# Autodesk Inventor assembly: drivetrain
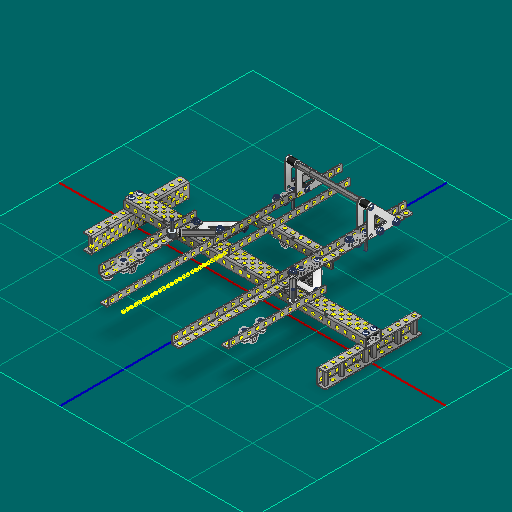
[picture p0: Inventor's stored thumbnail of the model, 512x512]
Saved by Autodesk Inventor 2025 (Build 290162000, 162)
## iProperties
Created: 2024-08-16
Part Number: drivetrain
Document SubType Name: Assembly
Designer: averey
Author: averey
## Documents named in this file (20)
- C:\Users\avere\vex_robotics_high_stakes\hardware\cad\ATLAS\chassis\structure\!structure.iam
- !structure.iam
- C:\Users\avere\vex_robotics_high_stakes\hardware\cad\ATLAS\chassis\structure\side_channel.iam
- C:\Users\avere\vex_robotics_high_stakes\hardware\cad\VEX-CAD-Inventor\Structure\Angle\Aluminum 1x1\Alu Angle 1x1x28.ipt
- C:\Users\avere\vex_robotics_high_stakes\hardware\cad\VEX-CAD-Inventor\Structure\C Channel\Aluminum 1x2x1\Alu C 1x2x1x30.ipt
- C:\Users\avere\vex_robotics_high_stakes\hardware\cad\ATLAS\chassis\structure\rail.iam
- C:\Users\avere\vex_robotics_high_stakes\hardware\cad\ATLAS\chassis\structure\rail_mirrored\rail_mirrored.iam
- C:\Users\avere\vex_robotics_high_stakes\hardware\cad\VEX-CAD-Inventor\Structure\Angle\Aluminum 1x1\Alu Angle 1x1x10.ipt
- C:\Users\avere\vex_robotics_high_stakes\hardware\cad\VEX-CAD-Inventor\Motion\Shaft LS\LS Pillow Bearing Block.ipt
- C:\Users\avere\vex_robotics_high_stakes\hardware\cad\VEX-CAD-Inventor\Motion\Spacers\Spacer Nylon .375 OD\NSpacer .375 OD x .375.ipt
- C:\Users\avere\vex_robotics_high_stakes\hardware\cad\VEX-CAD-Inventor\Motion\Spacers\Spacer Nylon .375 OD.ipt
- C:\Users\avere\vex_robotics_high_stakes\hardware\cad\VEX-CAD-Inventor\Motion\Spacers\Washer Teflon\TWasher .375 OD x .06250.ipt
- C:\Users\avere\vex_robotics_high_stakes\hardware\cad\VEX-CAD-Inventor\Motion\Spacers\Washer Teflon.ipt
- C:\Users\avere\vex_robotics_high_stakes\hardware\cad\VEX-CAD-Inventor\Structure\Hardware\Screw Steel - Star\SScrew Star Smooth .750.ipt
- C:\Users\avere\vex_robotics_high_stakes\hardware\cad\VEX-CAD-Inventor\Structure\Hardware\Screw Steel - Star.ipt
- C:\Users\avere\vex_robotics_high_stakes\hardware\cad\VEX-CAD-Inventor\Motion\Spacers\Spacer Nylon .500 OD\NSpacer White .500 OD x .125.ipt
- C:\Users\avere\vex_robotics_high_stakes\hardware\cad\VEX-CAD-Inventor\Motion\Spacers\Spacer Nylon .500 OD.ipt
- C:\Users\avere\vex_robotics_high_stakes\hardware\cad\VEX-CAD-Inventor\Structure\Standoff\Standoff .75.ipt
- C:\Users\avere\vex_robotics_high_stakes\hardware\cad\VEX-CAD-Inventor\Structure\Standoff.ipt
- C:\Users\avere\vex_robotics_high_stakes\hardware\cad\VEX-CAD-Inventor\Structure\Standoff\Standoff 3.00.ipt
## Components (19 placed, 13 different names)
1. side_channel:1 [sub-assembly] — Insert:83, Mate:44
2. side_channel:2 [sub-assembly] — Insert:82, Mate:43
3. Alu Angle 1x1x28:1
4. Alu C 1x2x1x30:1 — Insert:82, Mate:43, Insert:83, Mate:44, Insert:89, Mate:47, Insert:90, Mate:48, Mate:50, Insert:101, Insert:102, Insert:103, Insert:104
5. rail:1 [sub-assembly] — Insert:89, Mate:47, Mate:50, Mate:52, Insert:108
6. rail_mirrored:1 [sub-assembly] — Insert:90, Mate:48, Insert:92, Insert:105
7. Alu Angle 1x1x10:1 — Insert:92, Mate:52, Mate:53, Insert:100
8. LS Pillow Bearing Block:1 — Insert:98, Insert:99
9. NSpacer .375 OD x .375:1 — Insert:94, Insert:100
10. TWasher .375 OD x .06250:1 — Insert:94, Insert:99
11. TWasher .375 OD x .06250:2 — Insert:95, Insert:98
12. NSpacer .375 OD x .375:2 — Insert:95, Mate:53
13. SScrew Star Smooth .750:1 — Insert:101
14. SScrew Star Smooth .750:2 — Insert:102
15. SScrew Star Smooth .750:3 — Insert:103
16. SScrew Star Smooth .750:4 — Insert:104
17. NSpacer White .500 OD x .125:2 — Insert:105
18. Standoff .75:1 — Insert:107, Flush:1
19. Standoff 3.00:2 — Insert:107, Flush:1, Insert:108
## Relationships (25: Insert 17, Mate 7, Flush 1)
- Insert:82: side_channel:2 ↔ Alu C 1x2x1x30:1
- Mate:43: side_channel:2 ↔ Alu C 1x2x1x30:1
- Insert:83: side_channel:1 ↔ Alu C 1x2x1x30:1
- Mate:44: side_channel:1 ↔ Alu C 1x2x1x30:1
- Insert:89: Alu C 1x2x1x30:1 ↔ rail:1
- Mate:47: Alu C 1x2x1x30:1 ↔ rail:1
- Insert:90: Alu C 1x2x1x30:1 ↔ rail_mirrored:1
- Mate:48: Alu C 1x2x1x30:1 ↔ rail_mirrored:1
- Mate:50: Alu C 1x2x1x30:1 ↔ rail:1
- Insert:92: rail_mirrored:1 ↔ Alu Angle 1x1x10:1
- Mate:52: rail:1 ↔ Alu Angle 1x1x10:1
- Insert:94: NSpacer .375 OD x .375:1 ↔ TWasher .375 OD x .06250:1
- Insert:95: TWasher .375 OD x .06250:2 ↔ NSpacer .375 OD x .375:2
- Insert:98: LS Pillow Bearing Block:1 ↔ TWasher .375 OD x .06250:2
- Insert:99: LS Pillow Bearing Block:1 ↔ TWasher .375 OD x .06250:1
- Mate:53: Alu Angle 1x1x10:1 ↔ NSpacer .375 OD x .375:2
- Insert:100: Alu Angle 1x1x10:1 ↔ NSpacer .375 OD x .375:1
- Insert:101: Alu C 1x2x1x30:1 ↔ SScrew Star Smooth .750:1
- Insert:102: Alu C 1x2x1x30:1 ↔ SScrew Star Smooth .750:2
- Insert:103: Alu C 1x2x1x30:1 ↔ SScrew Star Smooth .750:3
- Insert:104: Alu C 1x2x1x30:1 ↔ SScrew Star Smooth .750:4
- Insert:105: rail_mirrored:1 ↔ NSpacer White .500 OD x .125:2
- Insert:107: Standoff .75:1 ↔ Standoff 3.00:2
- Flush:1: Standoff .75:1 ↔ Standoff 3.00:2
- Insert:108: rail:1 ↔ Standoff 3.00:2
